# Autodesk Inventor assembly: クランク
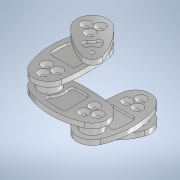
[picture p0: Inventor's stored thumbnail of the model, 180x180]
Saved by Autodesk Inventor 2022.2 (Build 262287010, 287A)
## iProperties
Created: 2022-01-08
Part Number: クランク
Document SubType Name: Assembly
Designer: acps
Author: acps
## Documents named in this file (5)
- C:\Users\acps\Documents\srdc\srdc_ksh\クランク.iam
- C:\Users\acps\Documents\srdc\srdc_ksh\カム\カム3.ipt
- C:\Users\acps\Documents\srdc\srdc_ksh\クランク\クランク_前.ipt
- C:\Users\acps\Documents\srdc\srdc_ksh\クランク\駆動節.ipt
- C:\Users\acps\Documents\srdc\srdc_ksh\クランク\クランク_中間.ipt
## Components (9 placed, 4 different names)
1. カム3:1 — Mate:3, Mate:4, Insert:2, Mate:17, Mate:18, Insert:9
2. カム3:2 — Mate:5, Mate:6, Insert:3, Mate:7, Mate:8, Insert:4
3. カム3:3 — Mate:9, Mate:10, Mate:11, Mate:12, Insert:6, Insert:10
4. クランク_前:1 — Mate:17, Mate:18, Insert:9
5. クランク_中間:1 — Mate:3, Mate:4, Insert:2, Mate:5, Mate:6, Insert:3
6. クランク_中間:2 — Mate:7, Mate:8, Insert:4, Mate:9, Mate:10, Insert:10
7. クランク_中間:3 — Mate:11, Mate:12, Insert:6, Mate:13, Mate:14, Insert:7
8. カム3:4 — Mate:13, Mate:14, Insert:7, Mate:15, Mate:16, Insert:8
9. 駆動節:1 — Mate:15, Mate:16, Insert:8
## Relationships (24: Mate 16, Insert 8)
- Mate:3: カム3:1 ↔ クランク_中間:1
- Mate:4: カム3:1 ↔ クランク_中間:1
- Insert:2: カム3:1 ↔ クランク_中間:1
- Mate:5: カム3:2 ↔ クランク_中間:1
- Mate:6: カム3:2 ↔ クランク_中間:1
- Insert:3: カム3:2 ↔ クランク_中間:1
- Mate:7: カム3:2 ↔ クランク_中間:2
- Mate:8: カム3:2 ↔ クランク_中間:2
- Insert:4: カム3:2 ↔ クランク_中間:2
- Mate:9: カム3:3 ↔ クランク_中間:2
- Mate:10: カム3:3 ↔ クランク_中間:2
- Mate:11: カム3:3 ↔ クランク_中間:3
- Mate:12: カム3:3 ↔ クランク_中間:3
- Insert:6: カム3:3 ↔ クランク_中間:3
- Mate:13: クランク_中間:3 ↔ カム3:4
- Mate:14: クランク_中間:3 ↔ カム3:4
- Insert:7: クランク_中間:3 ↔ カム3:4
- Mate:15: カム3:4 ↔ 駆動節:1
- Mate:16: カム3:4 ↔ 駆動節:1
- Insert:8: カム3:4 ↔ 駆動節:1
- Mate:17: カム3:1 ↔ クランク_前:1
- Mate:18: カム3:1 ↔ クランク_前:1
- Insert:9: カム3:1 ↔ クランク_前:1
- Insert:10: カム3:3 ↔ クランク_中間:2
